# Autodesk Inventor assembly: robot2
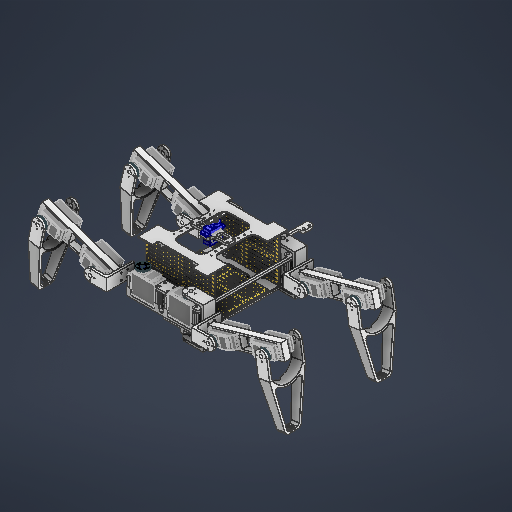
[picture p0: Inventor's stored thumbnail of the model, 512x512]
Saved by Autodesk Inventor 2026.1 (Build 301233000, 233)
## iProperties
Created: 2025-10-04
Part Number: robot2
Document SubType Name: Assembly
Designer: emanuel
Author: emanuel
## Documents named in this file (17)
- C:\Users\emanuel\UnFolder\SpiderRobo\3dmodel\robot3.iam
- C:\Users\emanuel\UnFolder\SpiderRobo\3dmodel\mg996r.ipt
- C:\Users\emanuel\UnFolder\SpiderRobo\3dmodel\support_2_servos.ipt
- C:\Users\emanuel\UnFolder\SpiderRobo\3dmodel\servo_disc.ipt
- C:\Users\emanuel\UnFolder\SpiderRobo\3dmodel\servo_support_4.ipt
- C:\Users\emanuel\UnFolder\SpiderRobo\3dmodel\C1.ipt
- C:\Users\emanuel\UnFolder\SpiderRobo\3dmodel\femur.ipt
- C:\Users\emanuel\UnFolder\SpiderRobo\3dmodel\L2.ipt
- C:\Users\emanuel\UnFolder\SpiderRobo\3dmodel\smart_calf.ipt
- C:\Users\emanuel\UnFolder\SpiderRobo\3dmodel\yellow_base.iam
- C:\Users\emanuel\UnFolder\SpiderRobo\3dmodel\base.ipt
- C:\Users\emanuel\UnFolder\SpiderRobo\3dmodel\sg90.ipt
- C:\Users\emanuel\UnFolder\SpiderRobo\3dmodel\microservo_support1.ipt
- C:\Users\emanuel\UnFolder\SpiderRobo\3dmodel\rigid_support1.ipt
- C:\Users\emanuel\UnFolder\SpiderRobo\3dmodel\rigid_support2.ipt
- C:\Users\emanuel\UnFolder\SpiderRobo\3dmodel\rigid_support3.ipt
- C:\Users\emanuel\UnFolder\SpiderRobo\3dmodel\battery1.ipt
## Components (63 placed, 16 different names)
1. support_2_servos:2 — Mate:20, Mate:21, Flush:6, Mate:22, Flush:7, Flush:8, Mate:23, Flush:9, Flush:10, Mate:24, Flush:11, Flush:12, Flush:33, Mate:147, Flush:34, Flush:49
2. mg996r:2 — Mate:40, Mate:41, Mate:42, Mate:204, Mate:205, Mate:206
3. servo_disc:2 — Mate:79, Mate:80
4. mg996r:3 — Mate:37, Mate:38, Mate:39
5. servo_disc:3 — Mate:69, Mate:70
6. servo_support_4:9 — Mate:20, Mate:21, Flush:6
7. servo_support_4:10 — Mate:23, Flush:9, Flush:10, Mate:37, Mate:38, Mate:39
8. servo_support_4:11 — Mate:22, Flush:7, Flush:8, Mate:40, Mate:41, Mate:42
9. servo_support_4:12 — Mate:24, Flush:11, Flush:12
10. L2:4 — Mate:71, Mate:72, Mate:73, Mate:121, Mate:122
11. C1:2 — Mate:69, Mate:70
12. L2:5 — Mate:123, Mate:124
13. C1:3 — Mate:71, Mate:72, Mate:73, Mate:79, Mate:80
14. mg996r:7
15. femur:2
16. servo_disc:7 — Mate:123, Mate:124
17. mg996r:8
18. servo_disc:8
19. smart_calf:2
20. mg996r:9
21. femur:3
22. servo_disc:9 — Mate:121, Mate:122
23. mg996r:10
24. servo_disc:10
25. smart_calf:3
26. base:1 — Mate:130, Mate:131, Mate:133, Mate:135, Mate:136, Mate:138, Flush:33, Mate:147, Flush:34, Flush:36, Flush:45, Mate:201, Flush:46, Mate:202, Flush:47, Mate:210, Flush:50
27. yellow_base:1 [sub-assembly] — Mate:130, Mate:131, Mate:139, Flush:37
28. yellow_base:2 [sub-assembly] — Mate:133, Mate:135, Flush:31, Mate:140, Flush:36
29. yellow_base:3 [sub-assembly] — Mate:136, Mate:138
30. base:2 — Mate:139, Flush:31, Mate:140, Mate:144, Mate:145, Mate:146, Flush:37
31. sg90:1 — Mate:141, Mate:142, Mate:143
32. microservo_support1:1 — Mate:141, Mate:142, Mate:143, Mate:144, Mate:145, Mate:146
33. support_2_servos:3 — Flush:45, Mate:201, Flush:46, Flush:48, Mate:211, Mate:212
34. mg996r:11 — Mate:209
35. servo_disc:11
36. mg996r:12 — Mate:207, Mate:208
37. servo_disc:12
38. servo_support_4:13
39. servo_support_4:14
40. servo_support_4:15
41. servo_support_4:16
42. L2:6
43. C1:4
44. L2:7
45. C1:5
46. mg996r:13
47. femur:4
48. servo_disc:13
49. mg996r:14
50. servo_disc:14
51. smart_calf:4
52. mg996r:15
53. femur:5
54. servo_disc:15
55. mg996r:16
56. servo_disc:16
57. smart_calf:5
58. rigid_support1:2 — Mate:202, Flush:47, Flush:48
59. rigid_support2:1 — Mate:204, Mate:205, Mate:206
60. rigid_support2:2
61. rigid_support3:1 — Mate:207, Mate:208, Mate:209
62. rigid_support1:3 — Mate:210, Mate:211, Mate:212, Mate:213
63. battery1:1 — Mate:213, Flush:49, Flush:50
## Relationships (158: Mate 133, Flush 25)
- [Mate]: mg996r:2 ↔ servo_disc:2
- [Mate]: mg996r:2 ↔ servo_disc:2
- [Mate]: mg996r:3 ↔ servo_disc:3
- [Mate]: mg996r:3 ↔ servo_disc:3
- Mate:20: support_2_servos:2 ↔ servo_support_4:9
- Mate:21: support_2_servos:2 ↔ servo_support_4:9
- Flush:6: support_2_servos:2 ↔ servo_support_4:9
- Mate:22: support_2_servos:2 ↔ servo_support_4:11
- Flush:7: support_2_servos:2 ↔ servo_support_4:11
- Flush:8: support_2_servos:2 ↔ servo_support_4:11
- Mate:23: support_2_servos:2 ↔ servo_support_4:10
- Flush:9: support_2_servos:2 ↔ servo_support_4:10
- Flush:10: support_2_servos:2 ↔ servo_support_4:10
- Mate:24: support_2_servos:2 ↔ servo_support_4:12
- Flush:11: support_2_servos:2 ↔ servo_support_4:12
- Flush:12: support_2_servos:2 ↔ servo_support_4:12
- Mate:37: mg996r:3 ↔ servo_support_4:10
- Mate:38: mg996r:3 ↔ servo_support_4:10
- Mate:39: mg996r:3 ↔ servo_support_4:10
- Mate:40: mg996r:2 ↔ servo_support_4:11
- Mate:41: mg996r:2 ↔ servo_support_4:11
- Mate:42: mg996r:2 ↔ servo_support_4:11
- [Mate]: C1:2 ↔ L2:5
- [Mate]: C1:2 ↔ L2:5
- [Mate]: C1:2 ↔ L2:5
- Mate:69: servo_disc:3 ↔ C1:2
- Mate:70: servo_disc:3 ↔ C1:2
- Mate:71: L2:4 ↔ C1:3
- Mate:72: L2:4 ↔ C1:3
- Mate:73: L2:4 ↔ C1:3
- Mate:79: servo_disc:2 ↔ C1:3
- Mate:80: servo_disc:2 ↔ C1:3
- [Mate]: mg996r:7 ↔ servo_disc:7
- [Mate]: mg996r:7 ↔ servo_disc:7
- [Mate]: mg996r:8 ↔ servo_disc:8
- [Mate]: mg996r:8 ↔ servo_disc:8
- [Mate]: mg996r:7 ↔ femur:2
- [Mate]: mg996r:7 ↔ femur:2
- [Mate]: mg996r:7 ↔ femur:2
- [Mate]: femur:2 ↔ mg996r:8
- [Mate]: femur:2 ↔ mg996r:8
- [Mate]: femur:2 ↔ mg996r:8
- [Mate]: servo_disc:8 ↔ smart_calf:2
- [Mate]: servo_disc:8 ↔ smart_calf:2
- [Mate]: mg996r:9 ↔ servo_disc:9
- [Mate]: mg996r:9 ↔ servo_disc:9
- [Mate]: mg996r:10 ↔ servo_disc:10
- [Mate]: mg996r:10 ↔ servo_disc:10
- [Mate]: mg996r:9 ↔ femur:3
- [Mate]: mg996r:9 ↔ femur:3
- [Mate]: mg996r:9 ↔ femur:3
- [Mate]: femur:3 ↔ mg996r:10
- [Mate]: femur:3 ↔ mg996r:10
- [Mate]: femur:3 ↔ mg996r:10
- [Mate]: servo_disc:10 ↔ smart_calf:3
- [Mate]: servo_disc:10 ↔ smart_calf:3
- Mate:121: L2:4 ↔ servo_disc:9
- Mate:122: L2:4 ↔ servo_disc:9
- Mate:123: L2:5 ↔ servo_disc:7
- Mate:124: L2:5 ↔ servo_disc:7
- Mate:130: base:1 ↔ yellow_base:1
- Mate:131: base:1 ↔ yellow_base:1
- Mate:133: base:1 ↔ yellow_base:2
- Mate:135: base:1 ↔ yellow_base:2
- Mate:136: base:1 ↔ yellow_base:3
- Mate:138: base:1 ↔ yellow_base:3
- Mate:139: yellow_base:1 ↔ base:2
- Flush:31: yellow_base:2 ↔ base:2
- Mate:140: yellow_base:2 ↔ base:2
- Mate:141: sg90:1 ↔ microservo_support1:1
- Mate:142: sg90:1 ↔ microservo_support1:1
- Mate:143: sg90:1 ↔ microservo_support1:1
- Mate:144: base:2 ↔ microservo_support1:1
- Mate:145: base:2 ↔ microservo_support1:1
- Mate:146: base:2 ↔ microservo_support1:1
- Flush:33: support_2_servos:2 ↔ base:1
- Mate:147: support_2_servos:2 ↔ base:1
- Flush:34: support_2_servos:2 ↔ base:1
- Flush:36: base:1 ↔ yellow_base:2
- Flush:37: yellow_base:1 ↔ base:2
- [Mate]: mg996r:11 ↔ servo_disc:11
- [Mate]: mg996r:11 ↔ servo_disc:11
- [Mate]: mg996r:12 ↔ servo_disc:12
- [Mate]: mg996r:12 ↔ servo_disc:12
- [Mate]: support_2_servos:3 ↔ servo_support_4:13
- [Mate]: support_2_servos:3 ↔ servo_support_4:13
- [Flush]: support_2_servos:3 ↔ servo_support_4:13
- [Mate]: support_2_servos:3 ↔ servo_support_4:15
- [Flush]: support_2_servos:3 ↔ servo_support_4:15
- [Flush]: support_2_servos:3 ↔ servo_support_4:15
- [Mate]: support_2_servos:3 ↔ servo_support_4:14
- [Flush]: support_2_servos:3 ↔ servo_support_4:14
- [Flush]: support_2_servos:3 ↔ servo_support_4:14
- [Mate]: support_2_servos:3 ↔ servo_support_4:16
- [Flush]: support_2_servos:3 ↔ servo_support_4:16
- [Flush]: support_2_servos:3 ↔ servo_support_4:16
- [Mate]: mg996r:12 ↔ servo_support_4:14
- [Mate]: mg996r:12 ↔ servo_support_4:14
- [Mate]: mg996r:12 ↔ servo_support_4:14
- [Mate]: mg996r:11 ↔ servo_support_4:15
- [Mate]: mg996r:11 ↔ servo_support_4:15
- [Mate]: mg996r:11 ↔ servo_support_4:15
- [Mate]: C1:4 ↔ L2:7
- [Mate]: C1:4 ↔ L2:7
- [Mate]: C1:4 ↔ L2:7
- [Mate]: servo_disc:12 ↔ C1:4
- [Mate]: servo_disc:12 ↔ C1:4
- [Mate]: L2:6 ↔ C1:5
- [Mate]: L2:6 ↔ C1:5
- [Mate]: L2:6 ↔ C1:5
- [Mate]: servo_disc:11 ↔ C1:5
- [Mate]: servo_disc:11 ↔ C1:5
- [Mate]: mg996r:13 ↔ servo_disc:13
- [Mate]: mg996r:13 ↔ servo_disc:13
- [Mate]: mg996r:14 ↔ servo_disc:14
- [Mate]: mg996r:14 ↔ servo_disc:14
- [Mate]: mg996r:13 ↔ femur:4
- [Mate]: mg996r:13 ↔ femur:4
- [Mate]: mg996r:13 ↔ femur:4
- [Mate]: femur:4 ↔ mg996r:14
- [Mate]: femur:4 ↔ mg996r:14
- [Mate]: femur:4 ↔ mg996r:14
- [Mate]: servo_disc:14 ↔ smart_calf:4
- [Mate]: servo_disc:14 ↔ smart_calf:4
- [Mate]: mg996r:15 ↔ servo_disc:15
- [Mate]: mg996r:15 ↔ servo_disc:15
- [Mate]: mg996r:16 ↔ servo_disc:16
- [Mate]: mg996r:16 ↔ servo_disc:16
- [Mate]: mg996r:15 ↔ femur:5
- [Mate]: mg996r:15 ↔ femur:5
- [Mate]: mg996r:15 ↔ femur:5
- [Mate]: femur:5 ↔ mg996r:16
- [Mate]: femur:5 ↔ mg996r:16
- [Mate]: femur:5 ↔ mg996r:16
- [Mate]: servo_disc:16 ↔ smart_calf:5
- [Mate]: servo_disc:16 ↔ smart_calf:5
- [Mate]: L2:6 ↔ servo_disc:15
- [Mate]: L2:6 ↔ servo_disc:15
- [Mate]: L2:7 ↔ servo_disc:13
- [Mate]: L2:7 ↔ servo_disc:13
- Flush:45: base:1 ↔ support_2_servos:3
- Mate:201: base:1 ↔ support_2_servos:3
- Flush:46: base:1 ↔ support_2_servos:3
- Mate:202: base:1 ↔ rigid_support1:2
- Flush:47: base:1 ↔ rigid_support1:2
- Flush:48: support_2_servos:3 ↔ rigid_support1:2
- Mate:204: mg996r:2 ↔ rigid_support2:1
- Mate:205: mg996r:2 ↔ rigid_support2:1
- Mate:206: mg996r:2 ↔ rigid_support2:1
- Mate:207: mg996r:12 ↔ rigid_support3:1
- Mate:208: mg996r:12 ↔ rigid_support3:1
- Mate:209: mg996r:11 ↔ rigid_support3:1
- Mate:210: base:1 ↔ rigid_support1:3
- Mate:211: support_2_servos:3 ↔ rigid_support1:3
- Mate:212: support_2_servos:3 ↔ rigid_support1:3
- Mate:213: rigid_support1:3 ↔ battery1:1
- Flush:49: support_2_servos:2 ↔ battery1:1
- Flush:50: base:1 ↔ battery1:1
## Named parameters: d49_d47 = 0 mm, d50_d48 = 0 mm, d51_d47 = 0 mm, d52_d48 = 0 mm, d138_d135 = 0 mm, d139_d136 = 0 mm, d140_d137 = 0 mm, d155_d153 = 0 mm, d156_d125 = 0 mm, d157_d126 = 0 mm, d158_d127_d125 = 0 mm, d159_d128_d126 = 0 mm, d160_d129 = 0 mm, d161_d130 = 0 mm, d162_d131 = 0 mm, d163_d132 = 0 mm, d164_d133 = 0 mm, d165_d134 = 0 mm, d166_d154 = 0 mm, d167_d153 = 0 mm, d168_d125 = 0 mm, d169_d126 = 0 mm, d170_d127_d125 = 0 mm, d171_d128_d126 = 0 mm, d172_d129 = 0 mm, d173_d130 = 0 mm, d174_d131 = 0 mm, d175_d132 = 0 mm, d176_d133 = 0 mm, d177_d134 = 0 mm, d178_d154 = 0 mm, d242_d193 = 0 mm, d243_d194 = 0 mm, d244_d195 = 0 mm, d245_d196 = 0 mm, d246_d144 = 0 mm, d247_d145 = 0 mm, d248_d151 = 0 mm, d249_d152 = 0 mm, d250_d155_d153 = 0 mm, d251_d156_d125 = 0 mm, d252_d157_d126 = 0 mm, d253_d158_d127_d125 = 0 mm, d254_d159_d128_d126 = 0 mm, d255_d160_d129 = 0 mm, d256_d161_d130 = 0 mm, d257_d162_d131 = 0 mm, d258_d163_d132 = 0 mm, d259_d164_d133 = 0 mm, d260_d165_d134 = 0 mm, d261_d166_d154 = 0 mm, d262_d167_d153 = 0 mm, d263_d168_d125 = 0 mm, d264_d169_d126 = 0 mm, d265_d170_d127_d125 = 0 mm, d266_d171_d128_d126 = 0 mm, d267_d172_d129 = 0 mm, d268_d173_d130 = 0 mm, d269_d174_d131 = 0 mm, d270_d175_d132 = 0 mm, d271_d176_d133 = 0 mm, d272_d177_d134 = 0 mm, d273_d178_d154 = 0 mm, d274_d138_d135 = 0 mm, d275_d139_d136 = 0 mm, d276_d140_d137 = 0 mm, d277_d141 = 0 mm, d278_d142 = 0 mm, d279_d143 = 0 mm, d280_d88 = 0 mm, d281_d89 = 0 mm, d282_d90 = 0 mm, d283_d91 = 0 mm, d284_d92 = 0 mm, d285_d93 = 0 mm, d286_d49_d47 = 0 mm, d287_d50_d48 = 0 mm, d288_d51_d47 = 0 mm, d289_d52_d48 = 0 mm, d290_d56 = 0 mm, d291_d57 = 0 mm, d292_d58 = 0 mm, d293_d59 = 0 mm, d294_d60 = 0 mm, d295_d61 = 0 mm, d296_d62 = 0 mm, d297_d63 = 0 mm, d298_d64 = 0 mm, d299_d65 = 0 mm, d300_d66 = 0 mm, d301_d67 = 0 mm
